# Autodesk Inventor assembly: Custom_Delta_Assembly
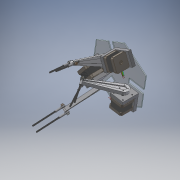
[picture p0: Inventor's stored thumbnail of the model, 180x180]
Saved by Autodesk Inventor 2019 (Build 230136000, 136)
## iProperties
Created: 2019-07-06
Part Number: Custom_Delta_Assembly
Document SubType Name: Assembly
Designer: Jorian Brusind
Author: Jorian Brusind
## Documents named in this file (10)
- C:\Users\Jorian Brusind\Documents\GitHub\ECE44x_Senior_Design\Design files\Delta Robot Arm\Inventor Files\Custom_Delta\Custom_Delta_Assembly.iam
- C:\Users\Jorian Brusind\Documents\GitHub\ECE44x_Senior_Design\Design files\Delta Robot Arm\Inventor Files\Custom_Delta\Stepper_Face.ipt
- C:\Users\Jorian Brusind\Documents\GitHub\ECE44x_Senior_Design\Design files\Delta Robot Arm\Inventor Files\nema-17-stepper-motor-with-v2-damper-1.snapshot.3\Nema 17  Stepper Motor length 34mm.ipt
- C:\Users\Jorian Brusind\Documents\GitHub\ECE44x_Senior_Design\Design files\Delta Robot Arm\Inventor Files\Stepper_Collar\products\12488\step\model.ipt
- C:\Users\Jorian Brusind\Documents\GitHub\ECE44x_Senior_Design\Design files\Delta Robot Arm\Inventor Files\Custom_Delta\Delta_Arm.ipt
- C:\Users\Jorian Brusind\Documents\GitHub\ECE44x_Senior_Design\Design files\Delta Robot Arm\Inventor Files\Custom_Delta\Delta_Top.ipt
- C:\Users\Jorian Brusind\Documents\GitHub\ECE44x_Senior_Design\Design files\Delta Robot Arm\Inventor Files\McMaster Files\59935K140_METRIC BALL JOINT ROD END.ipt
- C:\Users\Jorian Brusind\Documents\GitHub\ECE44x_Senior_Design\Design files\Delta Robot Arm\Inventor Files\Metric bolt\Bolt M4 40mm.ipt
- C:\Users\Jorian Brusind\Documents\GitHub\ECE44x_Senior_Design\Design files\Delta Robot Arm\Inventor Files\Metric nuts\Nut M4.ipt
- C:\Users\Jorian Brusind\Documents\GitHub\ECE44x_Senior_Design\Design files\Delta Robot Arm\Inventor Files\McMaster Files\94595A216_LOW-STRENGTH ZINC-PLATED STEEL THREADED ROD.ipt
## Components (31 placed, 9 different names)
1. Stepper_Face:1 — Mate:1, Mate:2, Mate:3, Mate:27, Mate:28, Mate:29
2. Nema 17  Stepper Motor length 34mm:1 — Mate:1, Mate:2, Mate:3, Mate:4, Flush:1
3. model:1 — Mate:4, Flush:1, Mate:7, Mate:8, Mate:9
4. Delta_Arm:1 — Mate:7, Mate:8, Flush:2, Mate:9, Mate:33, Mate:34, Mate:35, Mate:39
5. Stepper_Face:2 — Mate:30, Mate:31, Mate:32
6. Nema 17  Stepper Motor length 34mm:2
7. model:2
8. Delta_Arm:2 — Mate:43, Mate:44, Mate:45, Mate:46
9. Stepper_Face:3 — Mate:24, Mate:25, Mate:26
10. Nema 17  Stepper Motor length 34mm:3
11. model:3
12. Delta_Arm:3 — Mate:51, Mate:54, Mate:55
13. Delta_Top:1 — Mate:24, Mate:25, Mate:26, Mate:27, Mate:28, Mate:29, Mate:30, Mate:31, Mate:32
14. 59935K140_METRIC BALL JOINT ROD END:1 — Mate:35, Mate:37, Mate:38, Mate:40, Mate:65
15. 59935K140_METRIC BALL JOINT ROD END:2 — Mate:33, Mate:34, Mate:38, Mate:41, Mate:64
16. Bolt M4 40mm:1 — Mate:37, Mate:39, Mate:40, Mate:42
17. Nut M4:1 — Mate:41, Mate:42
18. Nut M4:2 — Mate:57, Mate:58
19. Nut M4:3 — Mate:49, Mate:50
20. Bolt M4 40mm:2 — Mate:47, Mate:48, Mate:49
21. Bolt M4 40mm:3 — Mate:51, Mate:52, Mate:53, Mate:56, Mate:57
22. 59935K140_METRIC BALL JOINT ROD END:3 — Mate:44, Mate:45, Mate:48, Mate:62, Mate:66
23. 59935K140_METRIC BALL JOINT ROD END:4 — Mate:43, Mate:46, Mate:47, Mate:50, Mate:63, Mate:67
24. 59935K140_METRIC BALL JOINT ROD END:5 — Mate:53, Mate:55, Mate:58, Mate:59, Mate:60
25. 59935K140_METRIC BALL JOINT ROD END:6 — Mate:52, Mate:54, Mate:56, Mate:61, Mate:68
26. 94595A216_LOW-STRENGTH ZINC-PLATED STEEL THREADED ROD:1 — Mate:64
27. 94595A216_LOW-STRENGTH ZINC-PLATED STEEL THREADED ROD:2 — Mate:63, Mate:67
28. 94595A216_LOW-STRENGTH ZINC-PLATED STEEL THREADED ROD:3 — Mate:65
29. 94595A216_LOW-STRENGTH ZINC-PLATED STEEL THREADED ROD:4 — Mate:61, Mate:68
30. 94595A216_LOW-STRENGTH ZINC-PLATED STEEL THREADED ROD:5 — Mate:62, Mate:66
31. 94595A216_LOW-STRENGTH ZINC-PLATED STEEL THREADED ROD:6 — Mate:59, Mate:60
## Relationships (69: Mate 65, Flush 4)
- Mate:1: Stepper_Face:1 ↔ Nema 17  Stepper Motor length 34mm:1
- Mate:2: Stepper_Face:1 ↔ Nema 17  Stepper Motor length 34mm:1
- Mate:3: Stepper_Face:1 ↔ Nema 17  Stepper Motor length 34mm:1
- Mate:4: Nema 17  Stepper Motor length 34mm:1 ↔ model:1
- Flush:1: Nema 17  Stepper Motor length 34mm:1 ↔ model:1
- Mate:7: model:1 ↔ Delta_Arm:1
- Mate:8: model:1 ↔ Delta_Arm:1
- Flush:2: Delta_Arm:1
- Mate:9: model:1 ↔ Delta_Arm:1
- [Mate]: Stepper_Face:2 ↔ Nema 17  Stepper Motor length 34mm:2
- [Mate]: Stepper_Face:2 ↔ Nema 17  Stepper Motor length 34mm:2
- [Mate]: Stepper_Face:2 ↔ Nema 17  Stepper Motor length 34mm:2
- [Mate]: Nema 17  Stepper Motor length 34mm:2 ↔ model:2
- [Flush]: Nema 17  Stepper Motor length 34mm:2 ↔ model:2
- [Mate]: model:2 ↔ Delta_Arm:2
- [Mate]: model:2 ↔ Delta_Arm:2
- [Mate]: model:2 ↔ Delta_Arm:2
- [Mate]: Stepper_Face:3 ↔ Nema 17  Stepper Motor length 34mm:3
- [Mate]: Stepper_Face:3 ↔ Nema 17  Stepper Motor length 34mm:3
- [Mate]: Stepper_Face:3 ↔ Nema 17  Stepper Motor length 34mm:3
- [Mate]: Nema 17  Stepper Motor length 34mm:3 ↔ model:3
- [Flush]: Nema 17  Stepper Motor length 34mm:3 ↔ model:3
- [Mate]: model:3 ↔ Delta_Arm:3
- [Mate]: model:3 ↔ Delta_Arm:3
- [Mate]: model:3 ↔ Delta_Arm:3
- Mate:24: Stepper_Face:3 ↔ Delta_Top:1
- Mate:25: Stepper_Face:3 ↔ Delta_Top:1
- Mate:26: Stepper_Face:3 ↔ Delta_Top:1
- Mate:27: Stepper_Face:1 ↔ Delta_Top:1
- Mate:28: Stepper_Face:1 ↔ Delta_Top:1
- Mate:29: Stepper_Face:1 ↔ Delta_Top:1
- Mate:30: Stepper_Face:2 ↔ Delta_Top:1
- Mate:31: Stepper_Face:2 ↔ Delta_Top:1
- Mate:32: Stepper_Face:2 ↔ Delta_Top:1
- Mate:33: Delta_Arm:1 ↔ 59935K140_METRIC BALL JOINT ROD END:2
- Mate:34 (1 mm): Delta_Arm:1 ↔ 59935K140_METRIC BALL JOINT ROD END:2
- Mate:35 (1 mm): Delta_Arm:1 ↔ 59935K140_METRIC BALL JOINT ROD END:1
- Mate:37: 59935K140_METRIC BALL JOINT ROD END:1 ↔ Bolt M4 40mm:1
- Mate:38: 59935K140_METRIC BALL JOINT ROD END:1 ↔ 59935K140_METRIC BALL JOINT ROD END:2
- Mate:39: Delta_Arm:1 ↔ Bolt M4 40mm:1
- Mate:40: 59935K140_METRIC BALL JOINT ROD END:1 ↔ Bolt M4 40mm:1
- Mate:41: 59935K140_METRIC BALL JOINT ROD END:2 ↔ Nut M4:1
- Mate:42: Bolt M4 40mm:1 ↔ Nut M4:1
- Mate:43: Delta_Arm:2 ↔ 59935K140_METRIC BALL JOINT ROD END:4
- Mate:44: Delta_Arm:2 ↔ 59935K140_METRIC BALL JOINT ROD END:3
- Mate:45 (1 mm): Delta_Arm:2 ↔ 59935K140_METRIC BALL JOINT ROD END:3
- Mate:46 (1 mm): Delta_Arm:2 ↔ 59935K140_METRIC BALL JOINT ROD END:4
- Mate:47: Bolt M4 40mm:2 ↔ 59935K140_METRIC BALL JOINT ROD END:4
- Mate:48: Bolt M4 40mm:2 ↔ 59935K140_METRIC BALL JOINT ROD END:3
- Mate:49: Nut M4:3 ↔ Bolt M4 40mm:2
- Mate:50: Nut M4:3 ↔ 59935K140_METRIC BALL JOINT ROD END:4
- Mate:51: Delta_Arm:3 ↔ Bolt M4 40mm:3
- Mate:52: Bolt M4 40mm:3 ↔ 59935K140_METRIC BALL JOINT ROD END:6
- Mate:53: Bolt M4 40mm:3 ↔ 59935K140_METRIC BALL JOINT ROD END:5
- Mate:54 (1 mm): Delta_Arm:3 ↔ 59935K140_METRIC BALL JOINT ROD END:6
- Mate:55 (1 mm): Delta_Arm:3 ↔ 59935K140_METRIC BALL JOINT ROD END:5
- Mate:56: Bolt M4 40mm:3 ↔ 59935K140_METRIC BALL JOINT ROD END:6
- Mate:57: Nut M4:2 ↔ Bolt M4 40mm:3
- Mate:58: Nut M4:2 ↔ 59935K140_METRIC BALL JOINT ROD END:5
- Mate:59: 59935K140_METRIC BALL JOINT ROD END:5 ↔ 94595A216_LOW-STRENGTH ZINC-PLATED STEEL THREADED ROD:6
- Mate:60: 59935K140_METRIC BALL JOINT ROD END:5 ↔ 94595A216_LOW-STRENGTH ZINC-PLATED STEEL THREADED ROD:6
- Mate:61: 59935K140_METRIC BALL JOINT ROD END:6 ↔ 94595A216_LOW-STRENGTH ZINC-PLATED STEEL THREADED ROD:4
- Mate:62: 59935K140_METRIC BALL JOINT ROD END:3 ↔ 94595A216_LOW-STRENGTH ZINC-PLATED STEEL THREADED ROD:5
- Mate:63: 59935K140_METRIC BALL JOINT ROD END:4 ↔ 94595A216_LOW-STRENGTH ZINC-PLATED STEEL THREADED ROD:2
- Mate:64: 59935K140_METRIC BALL JOINT ROD END:2 ↔ 94595A216_LOW-STRENGTH ZINC-PLATED STEEL THREADED ROD:1
- Mate:65: 59935K140_METRIC BALL JOINT ROD END:1 ↔ 94595A216_LOW-STRENGTH ZINC-PLATED STEEL THREADED ROD:3
- Mate:66: 59935K140_METRIC BALL JOINT ROD END:3 ↔ 94595A216_LOW-STRENGTH ZINC-PLATED STEEL THREADED ROD:5
- Mate:67: 59935K140_METRIC BALL JOINT ROD END:4 ↔ 94595A216_LOW-STRENGTH ZINC-PLATED STEEL THREADED ROD:2
- Mate:68: 59935K140_METRIC BALL JOINT ROD END:6 ↔ 94595A216_LOW-STRENGTH ZINC-PLATED STEEL THREADED ROD:4
## Named parameters: d13_d12 = 0 mm, d14_d5 = 0 mm, d15_d7 = 0 mm, d16_d8 = 0 mm, d17_d0 = 0 mm, d18_d1 = 0 mm, d19_d2 = 0 mm, d20_d3 = 0 mm, d21_d12 = 0 mm, d22_d5 = 0 mm, d23_d7 = 0 mm, d24_d8 = 0 mm, d25_d0 = 0 mm, d26_d1 = 0 mm, d27_d2 = 0 mm, d28_d3 = 0 mm
